# Autodesk Inventor assembly: COTS_IGUS_04_Series_Cable_Chain
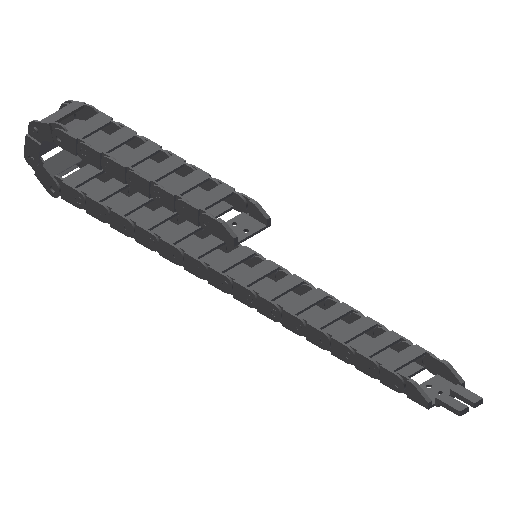
[picture p0: Inventor's stored thumbnail of the model, 512x512]
Saved by Autodesk Inventor 2026.1 (Build 301233000, 233)
## iProperties
Created: 2016-06-22
Part Number: COTS_IGUS_04_Series_Cable_Chain
Material: Ogólny
Document SubType Name: Assembly
Designer: Andrzej
Mass: 33.7172 g
Surface Area: 509.521 cm^2
Volume: 33.7172 cm^3
Density: 1 g/cm^3
Author: Andrzej
## Documents named in this file (5)
- C:\Users\Andrzej\OneDrive\_DRIVE_SYNCH_FILES\__ BYTECHLAB PROJECTS\MECH - FDM 3D Printer - RAPTOR-360\MCAD\1_REV1\__COTS_PARTS\COTS_IGUS_04_Series_Cable_Chain\COTS_IGUS_04_Series_Cable_Chain.iam
- C:\Users\Andrzej\OneDrive\_DRIVE_SYNCH_FILES\__ BYTECHLAB PROJECTS\MECH - FDM 3D Printer - RAPTOR-360\MCAD\1_REV1\__COTS_PARTS\COTS_IGUS_04_Series_Cable_Chain\0.4008m 04.20.015.0_1.ipt
- C:\Users\Andrzej\OneDrive\_DRIVE_SYNCH_FILES\__ BYTECHLAB PROJECTS\MECH - FDM 3D Printer - RAPTOR-360\MCAD\1_REV1\__COTS_PARTS\COTS_IGUS_04_Series_Cable_Chain\0.4008m 04.20.015.0_2.ipt
- C:\Users\Andrzej\OneDrive\_DRIVE_SYNCH_FILES\__ BYTECHLAB PROJECTS\MECH - FDM 3D Printer - RAPTOR-360\MCAD\1_REV1\__COTS_PARTS\COTS_IGUS_04_Series_Cable_Chain\sskeleton.ipt
- C:\Users\Andrzej\OneDrive\_DRIVE_SYNCH_FILES\__ BYTECHLAB PROJECTS\MECH - FDM 3D Printer - RAPTOR-360\MCAD\1_REV1\__COTS_PARTS\COTS_IGUS_04_Series_Cable_Chain\0.4008m 04.20.015.0.ipt
## Components (26 placed, 4 different names)
1. 0.4008m 04.20.015.0_1:1 — Równoległy:1, Kąt:1, Wstaw:1, Kąt:2
2. 0.4008m 04.20.015.0_2:1 — Równoległy:1, Kąt:1, Równoległy:2, Równoległy:3, Równoległy:4
3. sskeleton:1 — Równoległy:2, Równoległy:3, Równoległy:4
4. 0.4008m 04.20.015.0:1 — Wstaw:1, Kąt:2
5. 0.4008m 04.20.015.0:2
6. 0.4008m 04.20.015.0:3
7. 0.4008m 04.20.015.0:4
8. 0.4008m 04.20.015.0:5
9. 0.4008m 04.20.015.0:6
10. 0.4008m 04.20.015.0:7
11. 0.4008m 04.20.015.0:8
12. 0.4008m 04.20.015.0:9
13. 0.4008m 04.20.015.0:10
14. 0.4008m 04.20.015.0:11
15. 0.4008m 04.20.015.0:12
16. 0.4008m 04.20.015.0:13
17. 0.4008m 04.20.015.0:14
18. 0.4008m 04.20.015.0:15
19. 0.4008m 04.20.015.0:16
20. 0.4008m 04.20.015.0:17
21. 0.4008m 04.20.015.0:18
22. 0.4008m 04.20.015.0:19
23. 0.4008m 04.20.015.0:20
24. 0.4008m 04.20.015.0:21
25. 0.4008m 04.20.015.0:22
26. 0.4008m 04.20.015.0:23
## Component patterns: (23 elements, first: 0.4008m 04.20.015.0:1)
## Relationships (7: Flush 4, Angle 2, Insert 1)
- Równoległy:1 [Flush] (0.462 mm): 0.4008m 04.20.015.0_1:1 ↔ 0.4008m 04.20.015.0_2:1
- Kąt:1 [Angle] (0 deg): 0.4008m 04.20.015.0_1:1 ↔ 0.4008m 04.20.015.0_2:1
- Równoległy:2 [Flush]: 0.4008m 04.20.015.0_2:1 ↔ sskeleton:1
- Równoległy:3 [Flush]: 0.4008m 04.20.015.0_2:1 ↔ sskeleton:1
- Równoległy:4 [Flush]: 0.4008m 04.20.015.0_2:1 ↔ sskeleton:1
- Wstaw:1 [Insert]: 0.4008m 04.20.015.0_1:1 ↔ 0.4008m 04.20.015.0:1
- Kąt:2 [Angle] (0 deg): 0.4008m 04.20.015.0_1:1 ↔ 0.4008m 04.20.015.0:1
